# Autodesk Inventor assembly: 装配-载板
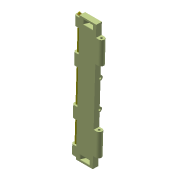
[picture p0: Inventor's stored thumbnail of the model, 180x180]
Saved by Autodesk Inventor 2015 (Build 190159000, 159)
## iProperties
Created: 2017-05-23
Part Number: 装配-载板
Document SubType Name: Assembly
Designer: Administrator
Author: Administrator
## Documents named in this file (4)
- C:\Users\Administrator\Desktop\毕设改终\装配-载板.iam
- C:\Users\Administrator\Desktop\毕设改终\载板连接销卡环.ipt
- C:\Users\Administrator\Desktop\毕设改终\载板.ipt
- C:\Users\Administrator\Desktop\毕设改终\载板连接销.ipt
## Components (4 placed, 3 different names)
1. 载板连接销卡环:1 — 配合:1, 相切:1
2. 载板连接销卡环:2 — 配合:2, 相切:2
3. 载板:1 — 插入:1, 相切:1, 相切:2
4. 载板连接销:1 — 插入:1, 配合:1, 配合:2
## Relationships (5: Mate 2, Tangent 2, Insert 1)
- 插入:1 [Insert]: 载板:1 ↔ 载板连接销:1
- 配合:1 [Mate]: 载板连接销卡环:1 ↔ 载板连接销:1
- 相切:1 [Tangent]: 载板连接销卡环:1 ↔ 载板:1
- 配合:2 [Mate]: 载板连接销卡环:2 ↔ 载板连接销:1
- 相切:2 [Tangent]: 载板连接销卡环:2 ↔ 载板:1
